# Autodesk Inventor assembly: Боковые стены
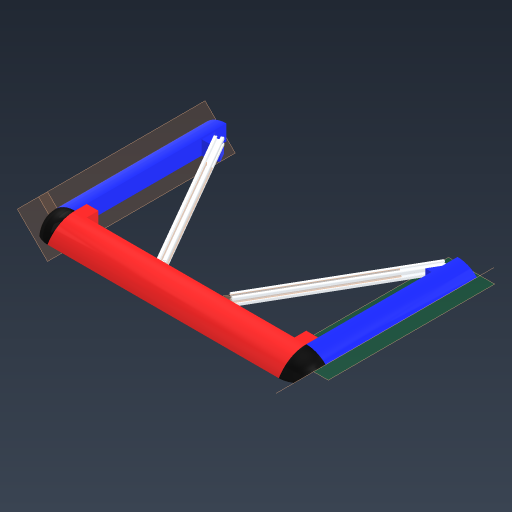
[picture p0: Inventor's stored thumbnail of the model, 512x512]
Saved by Autodesk Inventor 2023.2 (Build 272271030, 271C)
## iProperties
Created: 2025-08-19
Part Number: Боковые стены
Document SubType Name: Assembly
Designer: Олег Коноваленко
Author: Олег Коноваленко
## Documents named in this file (5)
- D:\!Rover\Rover\Rover_construction\Боковые стены.iam
- D:\!Rover\Rover\Rover_construction\Нижний край.ipt
- D:\!Rover\Rover\Rover_construction\пробник.ipt
- D:\!Rover\Rover\Rover_construction\Край стен.ipt
- D:\!Rover\Rover\Rover_construction\222LX-Konstruktsionnyy-profil-20kh20L.ipt
## Components (7 placed, 4 different names)
1. Нижний край:1 — Совмещение:7, Совмещение:13, Заподлицо:3, Совмещение:16, Совмещение:17, Совмещение:18, Совмещение:19, Совмещение:20, Совмещение:23
2. пробник:1 — Совмещение:7, Совмещение:13, Заподлицо:3, Совмещение:22
3. пробник:2 — Совмещение:16, Совмещение:17, Совмещение:18, Совмещение:21, Совмещение:24
4. Край стен:1 — Совмещение:20, Совмещение:21, Совмещение:24, Совмещение:27, Совмещение:28
5. Край стен:2 — Совмещение:19, Совмещение:22, Совмещение:23, Совмещение:25, Совмещение:26
6. 222LX-Konstruktsionnyy-profil-20kh20L:1 — Совмещение:27, Совмещение:28
7. 222LX-Konstruktsionnyy-profil-20kh20L:2 — Совмещение:25, Совмещение:26
## Relationships (16: Mate 15, Flush 1)
- Совмещение:7 [Mate]: Нижний край:1 ↔ пробник:1
- Совмещение:13 [Mate]: Нижний край:1 ↔ пробник:1
- Заподлицо:3 [Flush]: Нижний край:1 ↔ пробник:1
- Совмещение:16 [Mate]: Нижний край:1 ↔ пробник:2
- Совмещение:17 [Mate]: Нижний край:1 ↔ пробник:2
- Совмещение:18 [Mate]: Нижний край:1 ↔ пробник:2
- Совмещение:19 [Mate]: Нижний край:1 ↔ Край стен:2
- Совмещение:20 [Mate]: Нижний край:1 ↔ Край стен:1
- Совмещение:21 [Mate]: пробник:2 ↔ Край стен:1
- Совмещение:22 [Mate]: пробник:1 ↔ Край стен:2
- Совмещение:23 [Mate]: Нижний край:1 ↔ Край стен:2
- Совмещение:24 [Mate]: пробник:2 ↔ Край стен:1
- Совмещение:25 [Mate]: Край стен:2 ↔ 222LX-Konstruktsionnyy-profil-20kh20L:2
- Совмещение:26 [Mate]: Край стен:2 ↔ 222LX-Konstruktsionnyy-profil-20kh20L:2
- Совмещение:27 [Mate]: Край стен:1 ↔ 222LX-Konstruktsionnyy-profil-20kh20L:1
- Совмещение:28 [Mate]: Край стен:1 ↔ 222LX-Konstruktsionnyy-profil-20kh20L:1
